# Autodesk Inventor assembly: Exstra håndtag
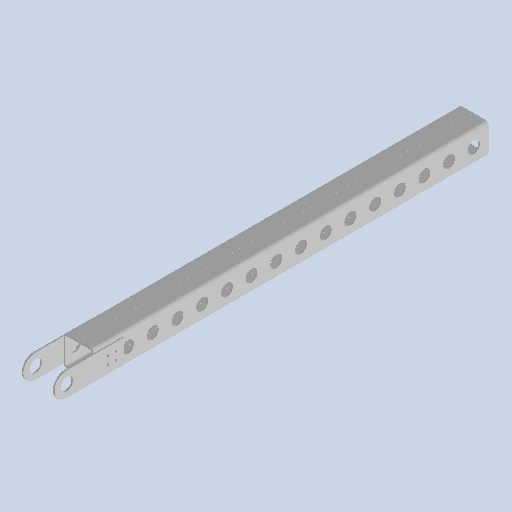
[picture p0: Inventor's stored thumbnail of the model, 512x512]
Saved by Autodesk Inventor 2022 (Build 260153000, 153)
## iProperties
Created: 2022-04-12
Part Number: Exstra håndtag
Document SubType Name: Weldment
Designer: Patrick
Weld Material: Welded Aluminum-6061
Author: Patrick
## Documents named in this file (3)
- C:\Users\patri\OneDrive - Syddansk Universitet\2. Semester Master\Mekaniske Elementer\Mini Project\2020-10-23\Workspaces\Workspace\Exstra håndtag.iam
- C:\Users\patri\OneDrive - Syddansk Universitet\2. Semester Master\Mekaniske Elementer\Mini Project\2020-10-23\Workspaces\Workspace\Extra led trækhåndtag.ipt
- C:\Users\patri\OneDrive - Syddansk Universitet\2. Semester Master\Mekaniske Elementer\Mini Project\2020-10-23\Workspaces\Workspace\Beslag ekstra håndtag.ipt
## Components (4 placed, 2 different names)
1. Extra led trækhåndtag:1 — Rigid:3, Rigid:4
2. Extra led trækhåndtag:2 — Rigid:2, Rigid:4
3. Beslag ekstra håndtag:1 — Rigid:3
4. Beslag ekstra håndtag:2 — Rigid:2
## Relationships (3: WeldJoint 3)
- Rigid:2 [WeldJoint]: Extra led trækhåndtag:2 ↔ Beslag ekstra håndtag:2
- Rigid:3 [WeldJoint]: Extra led trækhåndtag:1 ↔ Beslag ekstra håndtag:1
- Rigid:4 [WeldJoint]: Extra led trækhåndtag:1 ↔ Extra led trækhåndtag:2
